# Autodesk Inventor assembly: SEPARACION LATA-BOTELLA Y PAPEL
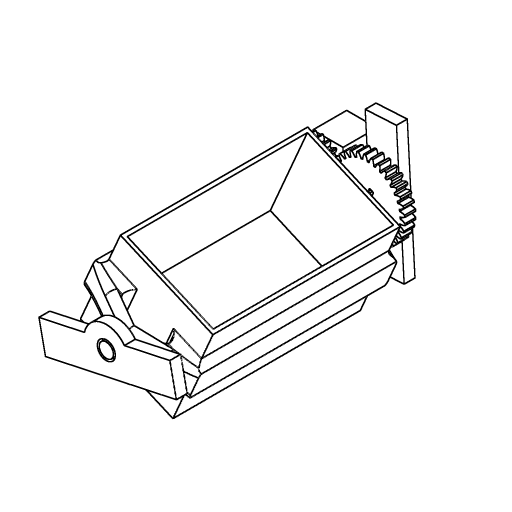
[picture p0: Inventor's stored thumbnail of the model, 512x512]
Saved by Autodesk Inventor 2024 (Build 280153000, 153)
## iProperties
Created: 2024-06-16
Part Number: SEPARACION LATA-BOTELLA Y PAPEL
Document SubType Name: Assembly
Designer: Jhuliams
Author: Jhuliams
## Documents named in this file (6)
- C:\Users\Jhuliams\Documents\GitHub\RECICLADOR_MODELO_3D\MECANISMO DE COMPACTADO\SEPARACION LATA-BOTELLA Y PAPEL.iam
- C:\Users\Jhuliams\Documents\GitHub\RECICLADOR_MODELO_3D\MECANISMO DE COMPACTADO\CAJA PARA DETECCION DE OBJETO.ipt
- C:\Users\Jhuliams\Documents\GitHub\RECICLADOR_MODELO_3D\MECANISMO DE COMPACTADO\ENGRANAJE CONDUCTOR DE CAJA.ipt
- C:\Users\Jhuliams\Documents\GitHub\RECICLADOR_MODELO_3D\MECANISMO DE COMPACTADO\ENGRANE MOTRIZ DE CAJA.ipt
- C:\Users\Jhuliams\Documents\GitHub\RECICLADOR_MODELO_3D\MECANISMO DE COMPACTADO\SOPORTE DE CAJA SEPARADORA.ipt
- C:\Users\Jhuliams\Documents\GitHub\RECICLADOR_MODELO_3D\MECANISMO DE COMPACTADO\NEMA 17 PARA TAPA PRINCIPAL.ipt
## Components (6 placed, 5 different names)
1. NEMA 17 PARA TAPA PRINCIPAL:1 — Mate:1, Mate:2
2. ENGRANE MOTRIZ DE CAJA:1 — Mate:1, Mate:2, Flush:1, Mate:3, Rotation:1
3. ENGRANAJE CONDUCTOR DE CAJA:1 — Flush:1, Mate:3, Mate:4, Rotation:1, Mate:5, Flush:2, Mate:6
4. CAJA PARA DETECCION DE OBJETO:1 — Mate:5, Flush:2, Mate:6, Flush:3, Mate:7, Mate:8, Flush:4
5. SOPORTE DE CAJA SEPARADORA:1 — Flush:3, Mate:7
6. SOPORTE DE CAJA SEPARADORA:2 — Mate:8, Flush:4
## Relationships (13: Mate 8, Flush 4, RelateRotation 1)
- Mate:1: NEMA 17 PARA TAPA PRINCIPAL:1 ↔ ENGRANE MOTRIZ DE CAJA:1
- Mate:2: NEMA 17 PARA TAPA PRINCIPAL:1 ↔ ENGRANE MOTRIZ DE CAJA:1
- Flush:1: ENGRANE MOTRIZ DE CAJA:1 ↔ ENGRANAJE CONDUCTOR DE CAJA:1
- Mate:3 (79.5 mm): ENGRANE MOTRIZ DE CAJA:1 ↔ ENGRANAJE CONDUCTOR DE CAJA:1
- Mate:4: ENGRANAJE CONDUCTOR DE CAJA:1
- Rotation:1 [RelateRotation] (0.6061 ul): ENGRANE MOTRIZ DE CAJA:1 ↔ ENGRANAJE CONDUCTOR DE CAJA:1
- Mate:5: ENGRANAJE CONDUCTOR DE CAJA:1 ↔ CAJA PARA DETECCION DE OBJETO:1
- Flush:2: ENGRANAJE CONDUCTOR DE CAJA:1 ↔ CAJA PARA DETECCION DE OBJETO:1
- Mate:6: ENGRANAJE CONDUCTOR DE CAJA:1 ↔ CAJA PARA DETECCION DE OBJETO:1
- Flush:3: CAJA PARA DETECCION DE OBJETO:1 ↔ SOPORTE DE CAJA SEPARADORA:1
- Mate:7: CAJA PARA DETECCION DE OBJETO:1 ↔ SOPORTE DE CAJA SEPARADORA:1
- Mate:8: CAJA PARA DETECCION DE OBJETO:1 ↔ SOPORTE DE CAJA SEPARADORA:2
- Flush:4: CAJA PARA DETECCION DE OBJETO:1 ↔ SOPORTE DE CAJA SEPARADORA:2
